# Autodesk Inventor assembly: LowerBody_MIR
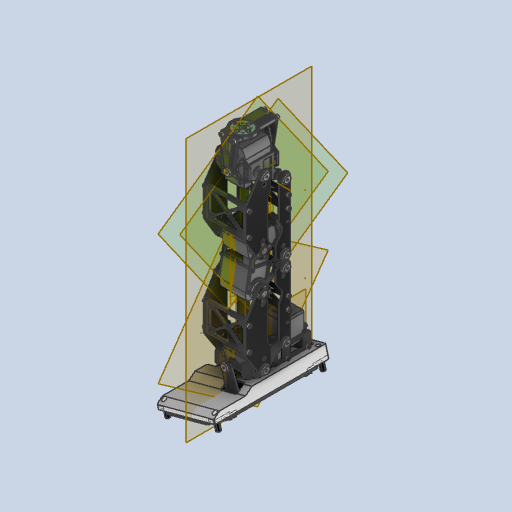
[picture p0: Inventor's stored thumbnail of the model, 512x512]
Saved by Autodesk Inventor 2022.5 (Build 265521000, 521)
## iProperties
Created: 2022-06-15
Part Number: LowerBody_MIR
Document SubType Name: Assembly
Designer: Masato Kubotera
Author: Masato Kubotera
## Documents named in this file (12)
- C:\Users\Masato\Documents\Inventor\SUSTAINA-OP\ModelingFiles\LowerBody\LowerBody_MIR.iam
- C:\Users\Masato\Documents\Inventor\SUSTAINA-OP\ModelingFiles\LowerBody\Leg_joint\Leg_joint_roll_yaw.iam
- C:\Users\Masato\Documents\Inventor\SUSTAINA-OP\ModelingFiles\LowerBody\Leg_joint\Leg_joint_roll_pitch.iam
- C:\Users\Masato\Documents\Inventor\SUSTAINA-OP\ModelingFiles\LowerBody\Slider_crank\Slider_crank_mechanism.iam
- C:\Users\Masato\Documents\Inventor\SUSTAINA-OP\ModelingFiles\LowerBody\Link\FrontLink.iam
- C:\Users\Masato\Documents\Inventor\SUSTAINA-OP\ModelingFiles\LowerBody\Link\BackUpperLink.iam
- C:\Users\Masato\Documents\Inventor\SUSTAINA-OP\ModelingFiles\LowerBody\Link\BackLowerLink.iam
- C:\Users\Masato\Documents\Inventor\SUSTAINA-OP\ModelingFiles\LowerBody\Knee\Knee_MIR.iam
- C:\Users\Masato\Documents\Inventor\SUSTAINA-OP\ModelingFiles\LowerBody\Ankle\Ankle_MIR.iam
- C:\Users\Masato\Documents\Inventor\SUSTAINA-OP\ModelingFiles\LowerBody\Foot\Foot_MIR.ipt
- C:\Users\Masato\Documents\Inventor\SUSTAINA-OP\ModelingFiles\LowerBody\Ankle\Ankle_independent_pitch.iam
- C:\Users\Masato\Documents\Inventor\SUSTAINA-OP\ModelingFiles\LowerBody\Foot\FootCover_MIR.iam
## Components (12 placed, 11 different names)
1. Leg_joint_roll_yaw:1 [sub-assembly] — 挿入:2, 挿入:1, フラッシュ:3, フラッシュ:2, フラッシュ:1, 付け根ロール軸, 付け根ロール軸:2
2. Leg_joint_roll_pitch:1 [sub-assembly] — 付け根ロール軸, 挿入:2, 挿入:1, 挿入:6, 挿入:5, 挿入:4, 挿入:3, 挿入:23
3. Slider_crank_mechanism:1 [sub-assembly] — 挿入:23, 付け根ロール軸:2
4. FrontLink:1 [sub-assembly] — 膝上ピッチ軸, 挿入:9, 挿入:7, 挿入:4, 挿入:3
5. BackUpperLink:1 [sub-assembly] — 挿入:10, 挿入:6, 挿入:5
6. Knee_MIR:1 [sub-assembly] — 挿入:14, 挿入:10, 膝上ピッチ軸, 挿入:9, 挿入:11, 挿入:13, 挿入:7, 挿入:12, 膝下ピッチ軸
7. BackLowerLink:1 [sub-assembly] — 挿入:14, 挿入:13, 挿入:22, 挿入:24
8. FrontLink:2 [sub-assembly] — 膝下ピッチ軸, 挿入:12, 挿入:11, 挿入:21, 挿入:23
9. Ankle_independent_pitch:1 [sub-assembly] — 挿入:21, 挿入:22, 挿入:23, 挿入:24, 挿入:25, 足首ピッチ軸
10. Ankle_MIR:1 [sub-assembly] — 足首ピッチ軸, 挿入:22, 挿入:21, 足首ロール軸, 挿入:25
11. Foot_MIR:1 — 挿入:22, 挿入:21, 足首ロール軸, Flush:3, Flush:4, Flush:5
12. FootCover_MIR:1 [sub-assembly] — Flush:3, Flush:4, Flush:5
## Relationships (33: Insert 21, Angle 6, Flush 5, Mate 1)
- 付け根ロール軸 [Angle] (180 deg): Leg_joint_roll_yaw:1 ↔ Leg_joint_roll_pitch:1
- 付け根ロール軸:2 [Angle] (0 deg): Leg_joint_roll_yaw:1 ↔ Slider_crank_mechanism:1
- 足首ロール軸 [Angle] (15 deg): Ankle_MIR:1 ↔ Foot_MIR:1
- 膝上ピッチ軸 [Angle] (180 deg): FrontLink:1 ↔ Knee_MIR:1
- 膝下ピッチ軸 [Angle] (0 deg): Knee_MIR:1 ↔ FrontLink:2
- 足首ピッチ軸 [Angle] (180 deg): Ankle_independent_pitch:1 ↔ Ankle_MIR:1
- 挿入:22 [Insert]: Ankle_MIR:1 ↔ Foot_MIR:1
- 挿入:21 [Insert]: Ankle_MIR:1 ↔ Foot_MIR:1
- 挿入:2 [Insert]: Leg_joint_roll_yaw:1 ↔ Leg_joint_roll_pitch:1
- 挿入:1 [Insert]: Leg_joint_roll_yaw:1 ↔ Leg_joint_roll_pitch:1
- フラッシュ:3 [Flush]: Leg_joint_roll_yaw:1
- フラッシュ:2 [Mate]: Leg_joint_roll_yaw:1
- フラッシュ:1 [Flush]: Leg_joint_roll_yaw:1
- 挿入:14 [Insert]: Knee_MIR:1 ↔ BackLowerLink:1
- 挿入:13 [Insert]: Knee_MIR:1 ↔ BackLowerLink:1
- 挿入:10 [Insert]: BackUpperLink:1 ↔ Knee_MIR:1
- 挿入:6 [Insert]: Leg_joint_roll_pitch:1 ↔ BackUpperLink:1
- 挿入:5 [Insert]: Leg_joint_roll_pitch:1 ↔ BackUpperLink:1
- 挿入:9 [Insert]: FrontLink:1 ↔ Knee_MIR:1
- 挿入:7 [Insert]: FrontLink:1 ↔ Knee_MIR:1
- 挿入:4 [Insert]: Leg_joint_roll_pitch:1 ↔ FrontLink:1
- 挿入:3 [Insert]: Leg_joint_roll_pitch:1 ↔ FrontLink:1
- 挿入:23 [Insert]: Leg_joint_roll_pitch:1 ↔ Slider_crank_mechanism:1
- 挿入:12 [Insert]: Knee_MIR:1 ↔ FrontLink:2
- 挿入:11 [Insert]: Knee_MIR:1 ↔ FrontLink:2
- 挿入:21 [Insert]: FrontLink:2 ↔ Ankle_independent_pitch:1
- 挿入:22 [Insert]: BackLowerLink:1 ↔ Ankle_independent_pitch:1
- 挿入:23 [Insert]: FrontLink:2 ↔ Ankle_independent_pitch:1
- 挿入:24 [Insert]: BackLowerLink:1 ↔ Ankle_independent_pitch:1
- 挿入:25 [Insert]: Ankle_independent_pitch:1 ↔ Ankle_MIR:1
- Flush:3: Foot_MIR:1 ↔ FootCover_MIR:1
- Flush:4: Foot_MIR:1 ↔ FootCover_MIR:1
- Flush:5: Foot_MIR:1 ↔ FootCover_MIR:1
